# Autodesk Inventor assembly: MKS Gen L with Standoffs
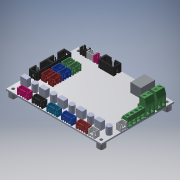
[picture p0: Inventor's stored thumbnail of the model, 180x180]
Saved by Autodesk Inventor 2019 (Build 230136000, 136)
## iProperties
Created: 2018-12-15
Part Number: MKS Gen L with Standoffs
Document SubType Name: Assembly
Designer: Ax
Author: Ax
## Documents named in this file (3)
- C:\Users\Ax\Google Drive\Inventor\Library\MKS Gen L with Standoffs.iam
- C:\Users\Ax\Google Drive\Inventor\Library\Makerbase.ipt
- C:\Users\Ax\Google Drive\Inventor\Library\lcd_spacer.ipt
## Components (5 placed, 2 different names)
1. Makerbase:1 — Mate:1, Mate:2, Flush:1, Rigid:1, Rigid:2, Rigid:3, Rigid:4
2. lcd_spacer:1 — Rigid:4
3. lcd_spacer:2 — Rigid:3
4. lcd_spacer:3 — Rigid:2
5. lcd_spacer:4 — Rigid:1
## Relationships (7: WeldJoint 4, Mate 2, Flush 1)
- Mate:1: Makerbase:1
- Mate:2: Makerbase:1
- Flush:1: Makerbase:1
- Rigid:1 [WeldJoint]: Makerbase:1 ↔ lcd_spacer:4
- Rigid:2 [WeldJoint]: Makerbase:1 ↔ lcd_spacer:3
- Rigid:3 [WeldJoint]: Makerbase:1 ↔ lcd_spacer:2
- Rigid:4 [WeldJoint]: Makerbase:1 ↔ lcd_spacer:1
